# Autodesk Inventor assembly: Assembly
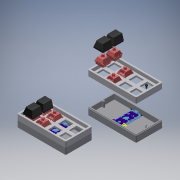
[picture p0: Inventor's stored thumbnail of the model, 180x180]
Saved by Autodesk Inventor 2018 (Build 220112000, 112)
## iProperties
Created: 2018-05-10
Part Number: Assembly
Document SubType Name: Assembly
Designer: mtsti
Author: mtsti
## Documents named in this file (7)
- C:\Users\mtsti\Desktop\Macro Deck\Assembly.iam
- C:\Users\mtsti\Desktop\Macro Deck\Arduino\Arduino Pro Micro Sparkfun.ipt
- C:\Users\mtsti\Desktop\Macro Deck\Switch\cherry old.ipt
- C:\Users\mtsti\Desktop\Macro Deck\Base.ipt
- C:\Users\mtsti\Desktop\Macro Deck\Key Plate.ipt
- C:\Users\mtsti\Desktop\Macro Deck\Keycap\MX 轴标准键帽.ipt
- C:\Users\mtsti\Desktop\Macro Deck\M2 Screw.ipt
## Components (21 placed, 6 different names)
1. Arduino Pro Micro Sparkfun:1 — Mate:20, Mate:21, Mate:22
2. cherry old:1 — Mate:5, Mate:6, Mate:7, Mate:11, Mate:12, Mate:13
3. cherry old:4 — Mate:17, Mate:18, Mate:19
4. cherry old:5 — Mate:14, Mate:15, Mate:16
5. cherry old:9 — Mate:2, Mate:3, Mate:4, Mate:8, Mate:9, Mate:10
6. Key Plate:1 — Mate:2, Mate:3, Mate:4, Mate:5, Mate:6, Mate:7, Mate:14, Mate:15, Mate:16, Mate:17, Mate:18, Mate:19, Mate:23, Flush:1, Flush:2, Mate:24, Mate:25, Mate:26, Mate:27
7. MX 轴标准键帽:1 — Mate:8, Mate:9, Mate:10
8. MX 轴标准键帽:2 — Mate:11, Mate:12, Mate:13
9. Base:2 — Mate:20, Mate:21, Mate:22, Mate:23, Flush:1, Flush:2
10. M2 Screw:1 — Mate:24, Mate:25
11. M2 Screw:2 — Mate:26, Mate:27
12. Arduino Pro Micro Sparkfun:2
13. cherry old:10
14. cherry old:11
15. cherry old:12
16. cherry old:13
17. Key Plate:2
18. MX 轴标准键帽:3
19. MX 轴标准键帽:4
20. Base:3
21. M2 Screw:4
## Relationships (54: Mate 50, Flush 4)
- Mate:2: cherry old:9 ↔ Key Plate:1
- Mate:3: cherry old:9 ↔ Key Plate:1
- Mate:4: cherry old:9 ↔ Key Plate:1
- Mate:5: cherry old:1 ↔ Key Plate:1
- Mate:6: cherry old:1 ↔ Key Plate:1
- Mate:7: cherry old:1 ↔ Key Plate:1
- Mate:8: cherry old:9 ↔ MX 轴标准键帽:1
- Mate:9: cherry old:9 ↔ MX 轴标准键帽:1
- Mate:10: cherry old:9 ↔ MX 轴标准键帽:1
- Mate:11: cherry old:1 ↔ MX 轴标准键帽:2
- Mate:12: cherry old:1 ↔ MX 轴标准键帽:2
- Mate:13: cherry old:1 ↔ MX 轴标准键帽:2
- Mate:14: cherry old:5 ↔ Key Plate:1
- Mate:15: cherry old:5 ↔ Key Plate:1
- Mate:16: cherry old:5 ↔ Key Plate:1
- Mate:17: cherry old:4 ↔ Key Plate:1
- Mate:18: cherry old:4 ↔ Key Plate:1
- Mate:19: cherry old:4 ↔ Key Plate:1
- Mate:20 (0.5 mm): Arduino Pro Micro Sparkfun:1 ↔ Base:2
- Mate:21 (-0.5 mm): Arduino Pro Micro Sparkfun:1 ↔ Base:2
- Mate:22: Arduino Pro Micro Sparkfun:1 ↔ Base:2
- Mate:23: Key Plate:1 ↔ Base:2
- Flush:1: Key Plate:1 ↔ Base:2
- Flush:2: Key Plate:1 ↔ Base:2
- Mate:24: Key Plate:1 ↔ M2 Screw:1
- Mate:25: Key Plate:1 ↔ M2 Screw:1
- Mate:26: Key Plate:1 ↔ M2 Screw:2
- Mate:27: Key Plate:1 ↔ M2 Screw:2
- [Mate] (20 mm): cherry old:13 ↔ Key Plate:2
- [Mate]: cherry old:13 ↔ Key Plate:2
- [Mate]: cherry old:13 ↔ Key Plate:2
- [Mate]: cherry old:10 ↔ Key Plate:2
- [Mate]: cherry old:10 ↔ Key Plate:2
- [Mate] (20 mm): cherry old:10 ↔ Key Plate:2
- [Mate] (15 mm): cherry old:13 ↔ MX 轴标准键帽:3
- [Mate]: cherry old:13 ↔ MX 轴标准键帽:3
- [Mate]: cherry old:13 ↔ MX 轴标准键帽:3
- [Mate] (15 mm): cherry old:10 ↔ MX 轴标准键帽:4
- [Mate]: cherry old:10 ↔ MX 轴标准键帽:4
- [Mate]: cherry old:10 ↔ MX 轴标准键帽:4
- [Mate]: cherry old:12 ↔ Key Plate:2
- [Mate]: cherry old:12 ↔ Key Plate:2
- [Mate]: cherry old:12 ↔ Key Plate:2
- [Mate]: cherry old:11 ↔ Key Plate:2
- [Mate]: cherry old:11 ↔ Key Plate:2
- [Mate]: cherry old:11 ↔ Key Plate:2
- [Mate] (0.5 mm): Arduino Pro Micro Sparkfun:2 ↔ Base:3
- [Mate] (-0.5 mm): Arduino Pro Micro Sparkfun:2 ↔ Base:3
- [Mate]: Arduino Pro Micro Sparkfun:2 ↔ Base:3
- [Mate] (50 mm): Key Plate:2 ↔ Base:3
- [Flush]: Key Plate:2 ↔ Base:3
- [Flush]: Key Plate:2 ↔ Base:3
- [Mate] (10 mm): Key Plate:2 ↔ M2 Screw:4
- [Mate]: Key Plate:2 ↔ M2 Screw:4
## Named parameters: d33_d3 = 20 mm, d34_d4 = 0 mm, d35_d5 = 0 mm, d36_d6 = 0 mm, d37_d7 = 0 mm, d38_d8 = 20 mm, d39_d9 = 15 mm, d40_d10 = 0 mm, d41_d11 = 0 mm, d42_d12 = 15 mm, d43_d13 = 0 mm, d44_d15 = 0 mm, d45_d16 = 0 mm, d46_d17 = 0 mm, d47_d18 = 0 mm, d48_d19 = 0 mm, d49_d20 = 0 mm, d50_d21 = 0 mm, d51_d22 = 0.5 mm, d52_d23 = -0.5 mm, d53_d25 = 0 mm, d54_d26 = 50 mm, d55_d27 = 0 mm, d56_d28 = 0 mm, d59_d31 = 10 mm, d60_d32 = 0 mm
